# Autodesk Inventor assembly: ASSEMBLY
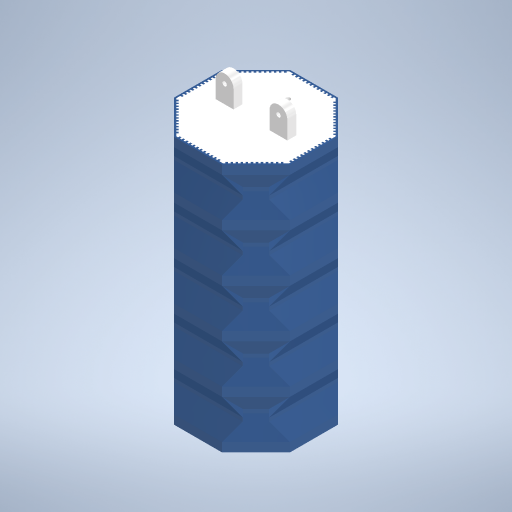
[picture p0: Inventor's stored thumbnail of the model, 512x512]
Saved by Autodesk Inventor 2024 (Build 280153000, 153)
## iProperties
Created: 2023-04-21
Part Number: ASSEMBLY
Document SubType Name: Assembly
Designer: didtk
Mass: 92.6531 g
Surface Area: 1183.77 cm^2
Volume: 92.6531 cm^3
Density: 1 g/cm^3
Author: didtk
## Documents named in this file (6)
- C:\승원\co-op\3rd_보근\Soft actuator\IPT,IAM\ASSEMBLY.iam
- C:\승원\co-op\3rd_보근\Soft actuator\IPT,IAM\pla_1layer(Z_0 최하단).ipt
- C:\승원\co-op\3rd_보근\Soft actuator\IPT,IAM\origami_linear actuator_octagon_V3(최하단).ipt
- C:\승원\co-op\3rd_보근\Soft actuator\IPT,IAM\origami_linear actuator_octagon_V3_1(중간-최상단).ipt
- C:\승원\co-op\3rd_보근\Soft actuator\IPT,IAM\pla 3(Z_37 중간 pla층).ipt
- C:\승원\co-op\3rd_보근\Soft actuator\IPT,IAM\pla_2(Z_64 최상단).ipt
## Components (11 placed, 5 different names)
1. pla_1layer(Z_0 최하단):1 — 플러쉬:1, 메이트:1, 메이트:2
2. origami_linear actuator_octagon_V3(최하단):1 — 플러쉬:1, 메이트:1, 메이트:2, 메이트:3, 메이트:4, 메이트:5, 메이트:6
3. pla_2(Z_64 최상단):1 — 메이트:7, 메이트:8
4. origami_linear actuator_octagon_V3_1(중간-최상단):1 — 메이트:3, 메이트:4, 메이트:5
5. origami_linear actuator_octagon_V3_1(중간-최상단):2
6. origami_linear actuator_octagon_V3_1(중간-최상단):3
7. origami_linear actuator_octagon_V3_1(중간-최상단):4 — 메이트:7, 메이트:8
8. pla 3(Z_37 중간 pla층):1 — 메이트:6
9. pla 3(Z_37 중간 pla층):2
10. pla 3(Z_37 중간 pla층):3
11. pla 3(Z_37 중간 pla층):4
## Component patterns: (4 elements, first: origami_linear actuator_octagon_V3_1(중간-최상단):1), (4 elements, first: pla 3(Z_37 중간 pla층):1)
## Relationships (9: Mate 8, Flush 1)
- 플러쉬:1 [Flush]: pla_1layer(Z_0 최하단):1 ↔ origami_linear actuator_octagon_V3(최하단):1
- 메이트:1 [Mate]: pla_1layer(Z_0 최하단):1 ↔ origami_linear actuator_octagon_V3(최하단):1
- 메이트:2 [Mate]: pla_1layer(Z_0 최하단):1 ↔ origami_linear actuator_octagon_V3(최하단):1
- 메이트:3 [Mate]: origami_linear actuator_octagon_V3(최하단):1 ↔ origami_linear actuator_octagon_V3_1(중간-최상단):1
- 메이트:4 [Mate]: origami_linear actuator_octagon_V3(최하단):1 ↔ origami_linear actuator_octagon_V3_1(중간-최상단):1
- 메이트:5 [Mate]: origami_linear actuator_octagon_V3(최하단):1 ↔ origami_linear actuator_octagon_V3_1(중간-최상단):1
- 메이트:6 [Mate]: origami_linear actuator_octagon_V3(최하단):1 ↔ pla 3(Z_37 중간 pla층):1
- 메이트:7 [Mate]: pla_2(Z_64 최상단):1 ↔ origami_linear actuator_octagon_V3_1(중간-최상단):4
- 메이트:8 [Mate]: pla_2(Z_64 최상단):1 ↔ origami_linear actuator_octagon_V3_1(중간-최상단):4
